# Autodesk Inventor assembly: Leg-40x
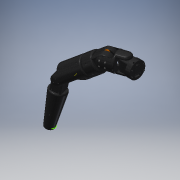
[picture p0: Inventor's stored thumbnail of the model, 180x180]
Saved by Autodesk Inventor 2018 (Build 220112000, 112)
## iProperties
Created: 2017-08-15
Part Number: Leg-40x
Material: Generisch
Document SubType Name: Assembly
Designer: JochenAlt
Author: JochenAlt
## Documents named in this file (9)
- D:\Projects\Manfred\design\cad\Inventor\Leg-40x.iam
- D:\Projects\Manfred\design\cad\Inventor\HipJoint-40x.ipt
- D:\Projects\Manfred\design\cad\Inventor\Thigh-40x.iam
- D:\Projects\Manfred\design\cad\Inventor\Rillenkugellager 11x7x3 inafag smr117.ipt
- D:\Projects\Manfred\design\cad\Inventor\Servobackaxis.ipt
- D:\Projects\Manfred\design\cad\Inventor\Foot-40x.iam
- D:\Projects\Manfred\design\cad\Inventor\Hip-40x.iam
- C:\Users\JochenAlt\Documents\Inventor\Content Center Files\R2018\de-DE\ISO 4762(1)\DIN EN ISO 4762 - M2 x 8.ipt
- C:\Users\JochenAlt\Documents\Inventor\Content Center Files\R2018\de-DE\ISO 4762(1)\DIN EN ISO 4762 - M2,5 x 4.ipt
## Components (17 placed, 8 different names)
1. HipJoint-40x:1 — Passend:34, Passend:35, Passend:36, Passend:37, Einfügen:1, Einfügen:2, Einfügen:3, Einfügen:4, Einfügen:5, Einfügen:6, Einfügen:7, Einfügen:8, Einfügen:9, Einfügen:10, Einfügen:11
2. Servobackaxis:1 — Passend:34, Passend:35, Passend:42, Passend:43
3. Rillenkugellager 11x7x3 inafag smr117:2 — Passend:36, Passend:37, Passend:38, Passend:39
4. Foot-40x:1 [sub-assembly] — Passend:40, Passend:41
5. Thigh-40x:1 [sub-assembly] — Passend:38, Passend:39, Passend:40, Passend:41
6. Hip-40x:1 [sub-assembly] — Passend:42, Passend:43
7. DIN EN ISO 4762 M2 x 8:4 — Einfügen:1
8. DIN EN ISO 4762 M2 x 8:3 — Einfügen:2
9. DIN EN ISO 4762 M2 x 8:2 — Einfügen:3
10. DIN EN ISO 4762 M2 x 8:1 — Einfügen:4
11. DIN EN ISO 4762 M2 x 8:7 — Einfügen:5
12. DIN EN ISO 4762 M2 x 8:6 — Einfügen:6
13. DIN EN ISO 4762 M2 x 8:5 — Einfügen:7
14. DIN EN ISO 4762 M2,5 x 4:2 — Einfügen:8
15. DIN EN ISO 4762 M2,5 x 4:3 — Einfügen:9
16. DIN EN ISO 4762 M2,5 x 4:4 — Einfügen:10
17. DIN EN ISO 4762 M2,5 x 4:1 — Einfügen:11
## Relationships (21: Insert 11, Mate 10)
- Passend:34 [Mate]: HipJoint-40x:1 ↔ Servobackaxis:1
- Passend:35 [Mate]: HipJoint-40x:1 ↔ Servobackaxis:1
- Passend:36 [Mate]: HipJoint-40x:1 ↔ Rillenkugellager 11x7x3 inafag smr117:2
- Passend:37 [Mate]: HipJoint-40x:1 ↔ Rillenkugellager 11x7x3 inafag smr117:2
- Passend:38 [Mate]: Rillenkugellager 11x7x3 inafag smr117:2 ↔ Thigh-40x:1
- Passend:39 [Mate]: Rillenkugellager 11x7x3 inafag smr117:2 ↔ Thigh-40x:1
- Passend:40 [Mate]: Foot-40x:1 ↔ Thigh-40x:1
- Passend:41 [Mate]: Foot-40x:1 ↔ Thigh-40x:1
- Passend:42 [Mate]: Servobackaxis:1 ↔ Hip-40x:1
- Passend:43 [Mate] (0.1 mm): Servobackaxis:1 ↔ Hip-40x:1
- Einfügen:1 [Insert]: HipJoint-40x:1 ↔ DIN EN ISO 4762 M2 x 8:4
- Einfügen:2 [Insert]: HipJoint-40x:1 ↔ DIN EN ISO 4762 M2 x 8:3
- Einfügen:3 [Insert]: HipJoint-40x:1 ↔ DIN EN ISO 4762 M2 x 8:2
- Einfügen:4 [Insert]: HipJoint-40x:1 ↔ DIN EN ISO 4762 M2 x 8:1
- Einfügen:5 [Insert]: HipJoint-40x:1 ↔ DIN EN ISO 4762 M2 x 8:7
- Einfügen:6 [Insert]: HipJoint-40x:1 ↔ DIN EN ISO 4762 M2 x 8:6
- Einfügen:7 [Insert]: HipJoint-40x:1 ↔ DIN EN ISO 4762 M2 x 8:5
- Einfügen:8 [Insert]: HipJoint-40x:1 ↔ DIN EN ISO 4762 M2,5 x 4:2
- Einfügen:9 [Insert]: HipJoint-40x:1 ↔ DIN EN ISO 4762 M2,5 x 4:3
- Einfügen:10 [Insert]: HipJoint-40x:1 ↔ DIN EN ISO 4762 M2,5 x 4:4
- Einfügen:11 [Insert]: HipJoint-40x:1 ↔ DIN EN ISO 4762 M2,5 x 4:1
